# Autodesk Inventor assembly: TestRig
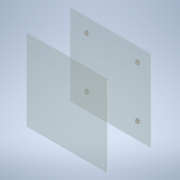
[picture p0: Inventor's stored thumbnail of the model, 180x180]
Saved by Autodesk Inventor 2020.3 (Build 243373010, 373A)
## iProperties
Created: 2020-10-30
Part Number: TestRig
Document SubType Name: Assembly
Designer: Naude Conradie
Author: Naude Conradie
## Documents named in this file (4)
- C:\Users\Naude Conradie\Desktop\Repository\Masters-Project\Models\Inventor\Testing Rig\TestRig.iam
- C:\Users\Naude Conradie\Desktop\Repository\Masters-Project\Models\Inventor\Testing Rig\Plate.ipt
- C:\Users\Naude Conradie\Desktop\Repository\Masters-Project\Models\Inventor\Testing Rig\PlateHoled.ipt
- C:\Users\Naude Conradie\Desktop\Repository\Masters-Project\Models\Inventor\Testing Rig\Plug.ipt
## Components (6 placed, 3 different names)
1. Plate:1 — Mate:4, Flush:3
2. PlateHoled:1 — Mate:4, Flush:3, Mate:6, Mate:7, Mate:8, Mate:9, Mate:10, Mate:11, Mate:12, Mate:13
3. Plug:1 — Mate:10, Mate:11
4. Plug:2 — Mate:12, Mate:13
5. Plug:3 — Mate:8, Mate:9
6. Plug:4 — Mate:6, Mate:7
## Relationships (10: Mate 9, Flush 1)
- Mate:4: Plate:1 ↔ PlateHoled:1
- Flush:3: Plate:1 ↔ PlateHoled:1
- Mate:6: PlateHoled:1 ↔ Plug:4
- Mate:7: PlateHoled:1 ↔ Plug:4
- Mate:8: PlateHoled:1 ↔ Plug:3
- Mate:9: PlateHoled:1 ↔ Plug:3
- Mate:10: PlateHoled:1 ↔ Plug:1
- Mate:11: PlateHoled:1 ↔ Plug:1
- Mate:12: PlateHoled:1 ↔ Plug:2
- Mate:13: PlateHoled:1 ↔ Plug:2
